# Autodesk Inventor assembly: Big Drill Complete
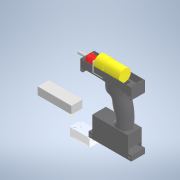
[picture p0: Inventor's stored thumbnail of the model, 180x180]
Saved by Autodesk Inventor 2022 (Build 260153000, 153)
## iProperties
Created: 2021-06-10
Part Number: Big Drill Complete
Document SubType Name: Assembly
Designer: jrcol
Author: jrcol
## Documents named in this file (6)
- C:\Users\jrcol\Desktop\Solar-Lab-Files\Smart Drill\Big Drill Complete.iam
- C:\Users\jrcol\Desktop\Solar-Lab-Files\Smart Drill\Big Housing C.ipt
- C:\Users\jrcol\Desktop\Solar-Lab-Files\Smart Drill\Big Shaft Motor Assembly.iam
- C:\Users\jrcol\Desktop\Solar-Lab-Files\Smart Drill\micro controller.ipt
- C:\Users\jrcol\Desktop\Solar-Lab-Files\Smart Drill\Battery.ipt
- C:\Users\jrcol\Desktop\Solar-Lab-Files\Smart Drill\Big Socket Extension.ipt
## Components (5 placed, 5 different names)
1. Big Socket Extension:2 — Mate:2
2. Big Housing C:1 — Mate:1, Mate:3
3. Big Shaft Motor Assembly:1 [sub-assembly] — Mate:1, Mate:2, Mate:3
4. micro controller:1
5. Battery:1
## Relationships (3: Mate 3)
- Mate:1: Big Housing C:1 ↔ Big Shaft Motor Assembly:1
- Mate:2: Big Socket Extension:2 ↔ Big Shaft Motor Assembly:1
- Mate:3 (5 mm): Big Housing C:1 ↔ Big Shaft Motor Assembly:1
